# Autodesk Inventor assembly: Assembly1
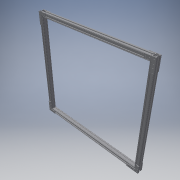
[picture p0: Inventor's stored thumbnail of the model, 180x180]
Saved by Autodesk Inventor 2018 (Build 220112000, 112)
## iProperties
Created: 2017-10-30
Part Number: Assembly1
Document SubType Name: Assembly
Designer: matts
Author: matts
## Documents named in this file (5)
- C:\Users\matts\Documents\Inventor\FTC 2018\Assembly1.iam
- C:\Users\matts\Documents\Inventor\Actobotics\All STEP Files\565 Parts\565062.ipt
- C:\Users\matts\Documents\Inventor\Actobotics\All STEP Files\585 parts\585076.ipt
- C:\Users\matts\Documents\Inventor\Actobotics\All STEP Files\565 Parts\565062_CPY.ipt
- C:\Users\matts\Documents\Inventor\Actobotics\All STEP Files\585 parts\585076_CPY.ipt
## Components (12 placed, 4 different names)
1. 565062:1 — Mate:1, Flush:1, Flush:2, Flush:3, Flush:4, Flush:6, Mate:7, Flush:13, Flush:14, Flush:19, Flush:21, Flush:22
2. 565062:2 — Mate:1, Flush:1, Flush:2, Mate:2, Mate:3, Flush:5, Mate:8, Flush:18
3. 585076:1 — Mate:2, Flush:3, Flush:4
4. 585076:2 — Mate:3, Flush:5, Flush:6
5. 565062_CPY:1 — Flush:7, Flush:8, Mate:4, Flush:9, Flush:10, Flush:11, Flush:15, Flush:16, Mate:9, Flush:17
6. 565062_CPY:2 — Flush:7, Flush:8, Mate:4, Mate:5, Flush:12, Mate:6, Mate:7, Flush:13, Flush:14, Mate:10, Flush:20, Mate:11
7. 585076_CPY:1 — Flush:9, Flush:10, Mate:5
8. 585076_CPY:2 — Flush:11, Flush:12, Mate:6
9. 585076:3 — Mate:8, Flush:15, Flush:16
10. 585076:4 — Mate:9, Flush:17, Flush:18
11. 585076:5 — Mate:10, Flush:19, Flush:20
12. 585076:6 — Mate:11, Flush:21, Flush:22
## Relationships (33: Flush 22, Mate 11)
- Mate:1: 565062:1 ↔ 565062:2
- Flush:1: 565062:1 ↔ 565062:2
- Flush:2: 565062:1 ↔ 565062:2
- Mate:2: 565062:2 ↔ 585076:1
- Flush:3: 565062:1 ↔ 585076:1
- Flush:4: 565062:1 ↔ 585076:1
- Mate:3: 565062:2 ↔ 585076:2
- Flush:5: 565062:2 ↔ 585076:2
- Flush:6: 565062:1 ↔ 585076:2
- Flush:7: 565062_CPY:1 ↔ 565062_CPY:2
- Flush:8: 565062_CPY:1 ↔ 565062_CPY:2
- Mate:4: 565062_CPY:1 ↔ 565062_CPY:2
- Flush:9: 565062_CPY:1 ↔ 585076_CPY:1
- Flush:10: 565062_CPY:1 ↔ 585076_CPY:1
- Mate:5: 565062_CPY:2 ↔ 585076_CPY:1
- Flush:11: 565062_CPY:1 ↔ 585076_CPY:2
- Flush:12: 565062_CPY:2 ↔ 585076_CPY:2
- Mate:6: 565062_CPY:2 ↔ 585076_CPY:2
- Mate:7: 565062:1 ↔ 565062_CPY:2
- Flush:13: 565062:1 ↔ 565062_CPY:2
- Flush:14: 565062:1 ↔ 565062_CPY:2
- Mate:8: 565062:2 ↔ 585076:3
- Flush:15: 565062_CPY:1 ↔ 585076:3
- Flush:16: 565062_CPY:1 ↔ 585076:3
- Mate:9: 565062_CPY:1 ↔ 585076:4
- Flush:17: 565062_CPY:1 ↔ 585076:4
- Flush:18: 565062:2 ↔ 585076:4
- Mate:10: 565062_CPY:2 ↔ 585076:5
- Flush:19: 565062:1 ↔ 585076:5
- Flush:20: 565062_CPY:2 ↔ 585076:5
- Mate:11: 565062_CPY:2 ↔ 585076:6
- Flush:21: 565062:1 ↔ 585076:6
- Flush:22: 565062:1 ↔ 585076:6
